# Autodesk Inventor assembly: Ensamble_Carcasa4.0
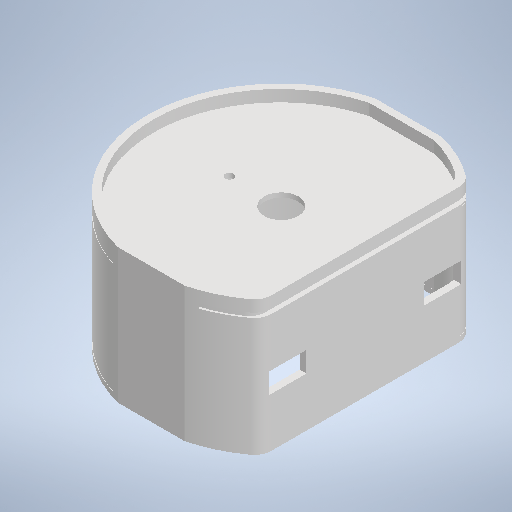
[picture p0: Inventor's stored thumbnail of the model, 512x512]
Saved by Autodesk Inventor 2025.3 (Build 293356030, 356C)
## iProperties
Created: 2025-10-09
Part Number: Ensamble_Carcasa4.0
Document SubType Name: Assembly
Designer: brene
Author: brene
## Documents named in this file (3)
- D:\OneDrive - Estudiantes ITCR\Documentos\GitHub\Atta-Bot-STEM\Chasis\Rediseño_Diego&Carlos\Carcasa 4.0 Rediseño\Ensamble_Carcasa4.0.iam
- D:\OneDrive - Estudiantes ITCR\Documentos\GitHub\Atta-Bot-STEM\Chasis\Rediseño_Diego&Carlos\Carcasa 4.0 Rediseño\carcasa4.0.ipt
- D:\OneDrive - Estudiantes ITCR\Documentos\GitHub\Atta-Bot-STEM\Chasis\Rediseño_Diego&Carlos\Carcasa 4.0 Rediseño\tapa_carcasa_4.0.ipt
## Components (2 placed, 2 different names)
1. carcasa4.0:1 — Mate:1
2. tapa_carcasa_4.0:1 — Mate:1
## Relationships (1: Mate 1)
- Mate:1: carcasa4.0:1 ↔ tapa_carcasa_4.0:1
